# Autodesk Inventor assembly: CoreXY Motor Assembly Right for 4040 - V3
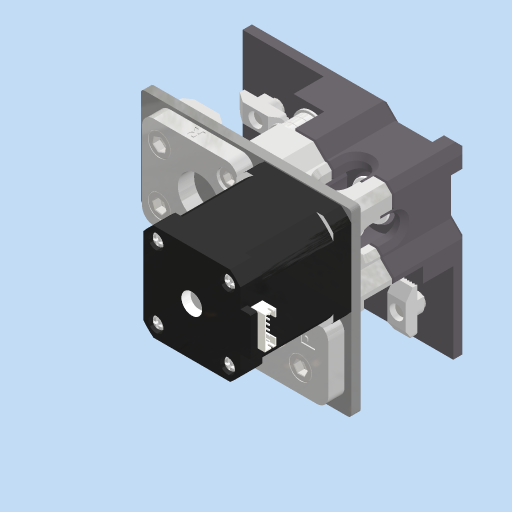
[picture p0: Inventor's stored thumbnail of the model, 512x512]
Saved by Autodesk Inventor 2023.2 (Build 272271000, 271)
## iProperties
Created: 2023-11-27
Part Number: CoreXY Motor Assembly Right for 4040 - V3
Document SubType Name: Assembly
Designer: Nils Bade
Author: Nils Bade
## Documents named in this file (17)
- C:\Users\nilsb\Documents\Inventor\Projektarbeit-Bade\RatRig_Bade\CoreXY Motor Assembly Right for 4040 - V3.iam
- C:\Users\nilsb\Documents\Inventor\Projektarbeit-Bade\RatRig_modified\Motor Plate Top for 4040.ipt
- C:\Users\nilsb\Documents\Inventor\Projektarbeit-Bade\RatRig_Standards\Nema 17 Stepper Motor - 48mm - 1.8degree_step, 76oz-in v1.ipt
- C:\Users\nilsb\Documents\Inventor\Projektarbeit-Bade\Schrauben\Cap Head Screw M3x35 v2.ipt
- C:\Users\nilsb\Documents\Inventor\Projektarbeit-Bade\RatRig_Standards\Timing Pulley - 2GT (2mm) - 20 Tooth - For 9mm Belt - 5mm Bo v1.ipt
- C:\Users\nilsb\Documents\Inventor\Projektarbeit-Bade\RatRig_modified\T-NUT - DropIn 4040 SERIES - M6.ipt
- C:\Users\nilsb\Documents\Inventor\Projektarbeit-Bade\Schrauben\Countersink Screw M6x14 v2.ipt
- C:\Users\nilsb\Documents\Inventor\Projektarbeit-Bade\Schrauben\Cap Head Screw M6x16.ipt
- C:\Users\nilsb\Documents\Inventor\Projektarbeit-Bade\RatRig_modified\xy Motor Support Left for 4040.ipt
- C:\Users\nilsb\Documents\Inventor\Projektarbeit-Bade\Schrauben\Cap Head Screw M5x40 v2.ipt
- C:\Users\nilsb\Documents\Inventor\Projektarbeit-Bade\RatRig_Standards\Hex Locking Nut - M5 v2.ipt
- C:\Users\nilsb\Documents\Inventor\Projektarbeit-Bade\RatRig_Standards\Mini Precision Shim - 8x5x1mm v2.ipt
- C:\Users\nilsb\Documents\Inventor\Projektarbeit-Bade\RatRig_Standards\Ball Bearing - F695ZZ v1.ipt
- C:\Users\nilsb\Documents\Inventor\Projektarbeit-Bade\RatRig_Standards\Ball Bearing - 695ZZ v1.ipt
- C:\Users\nilsb\Documents\Inventor\Projektarbeit-Bade\RatRig_modified\xy Motorcage Top Right for 4040 V2.ipt
- C:\Users\nilsb\Documents\Inventor\Projektarbeit-Bade\RatRig_modified\xy_motor_cage_bottom_right_v4.ipt
- C:\Users\nilsb\Documents\Inventor\Projektarbeit-Bade\RatRig_modified\xy Motor Support Right for 4040 extra.ipt
## Components (43 placed, 16 different names)
1. xy Motorcage Top Right for 4040 V2:2 — Passend:87
2. xy_motor_cage_bottom_right_v4:1 — Passend:87
3. Motor Plate Top for 4040:1 — Winkel:1, Passend:8, Passend:21, Passend:22, Passend:24, Passend:25, Winkel:5, Winkel:6, Winkel:7, Winkel:8, Passend:27, Passend:28, Passend:29, Passend:30, Passend:45, Passend:46, Passend:47, Passend:50, Passend:51, Passend:63, Passend:88, Passend:89, Passend:90, Passend:91, Passend:92, Passend:94
4. Nema 17 Stepper Motor - 48mm - 1.8degree_step, 76oz-in v1:1 — Winkel:1, Passend:8, Winkel:2, Passend:86
5. Cap Head Screw M3x35 v2:1
6. Cap Head Screw M3x35 v2:2
7. Cap Head Screw M3x35 v2:3
8. Cap Head Screw M3x35 v2:4
9. Timing Pulley - 2GT (2mm) - 20 Tooth - For 9mm Belt - 5mm Bo v1:1 — Winkel:2, Fluchtend:1, Passend:86
10. T-NUT - DROP IN TYPE FOR 40 SERIES - M6:1 — Passend:24, Winkel:7, Passend:28
11. T-NUT - DROP IN TYPE FOR 40 SERIES - M6:2 — Passend:25, Winkel:8, Passend:27
12. T-NUT - DROP IN TYPE FOR 40 SERIES - M6:3 — Passend:21, Winkel:5, Passend:30
13. T-NUT - DROP IN TYPE FOR 40 SERIES - M6:4 — Passend:22, Winkel:6, Passend:29, Passend:93
14. T-NUT - DROP IN TYPE FOR 40 SERIES - M6:5
15. T-NUT - DROP IN TYPE FOR 40 SERIES - M6:6
16. T-NUT - DROP IN TYPE FOR 40 SERIES - M6:7
17. Countersink Screw M6x14 v2:1
18. Countersink Screw M6x14 v2:2
19. Countersink Screw M6x14 v2:3
20. Cap Head Screw M6x16:1 — Passend:94, Passend:98
21. Cap Head Screw M6x16:2 — Passend:93, Passend:97
22. Cap Head Screw M6x16:3 — Passend:91, Passend:95
23. Cap Head Screw M6x16:4 — Passend:92, Passend:96
24. xy Motor Support Right for 4040 V2:1 — Passend:45, Passend:46, Passend:47, Passend:52, Passend:53, Passend:95, Passend:96
25. Cap Head Screw M5x40 v2:1 — Passend:50, Passend:53, Passend:54, Passend:58, Passend:59, Passend:67, Passend:69, Passend:71
26. Cap Head Screw M5x40 v2:2 — Passend:51, Passend:52, Passend:55, Passend:62, Passend:64, Passend:65, Passend:73, Passend:75, Passend:77, Passend:80, Passend:82, Passend:84
27. Hex Locking Nut - M5 v2:1 — Passend:55
28. Hex Locking Nut - M5 v2:2 — Passend:54
29. Mini Precision Shim - 8x5x1mm v2:1 — Passend:65, Passend:85
30. Mini Precision Shim - 8x5x1mm v2:2 — Passend:64, Passend:79, Passend:81
31. Mini Precision Shim - 8x5x1mm v2:3 — Passend:62, Passend:63, Passend:74
32. Mini Precision Shim - 8x5x1mm v2:4 — Passend:59, Passend:72
33. Mini Precision Shim - 8x5x1mm v2:5 — Passend:58, Passend:68
34. Ball Bearing - F695ZZ v1:1 — Passend:84, Passend:85, Fluchtend:1
35. Ball Bearing - F695ZZ v1:2 — Passend:77, Passend:78, Passend:79
36. Ball Bearing - F695ZZ v1:3 — Passend:71, Passend:72
37. Ball Bearing - F695ZZ v1:4 — Passend:80, Passend:81, Passend:83
38. Ball Bearing - F695ZZ v1:5 — Passend:73, Passend:74, Passend:76
39. Ball Bearing - F695ZZ v1:6 — Passend:67, Passend:68, Passend:70
40. Ball Bearing - 695ZZ v1:1 — Passend:82, Passend:83
41. Ball Bearing - 695ZZ v1:2 — Passend:75, Passend:76, Passend:78
42. Ball Bearing - 695ZZ v1:3 — Passend:69, Passend:70
43. xy Motor Support Right extra:1 — Passend:88, Passend:89, Passend:90, Passend:97, Passend:98
## Relationships (99: Mate 87, Angle 11, Flush 1)
- [Mate]: xy Motorcage Top Right for 4040 V2:2 ↔ xy_motor_cage_bottom_right_v4:1
- [Mate]: xy Motorcage Top Right for 4040 V2:2 ↔ xy_motor_cage_bottom_right_v4:1
- [Mate]: xy_motor_cage_bottom_right_v4:1 ↔ Motor Plate Top for 4040:1
- [Mate]: xy_motor_cage_bottom_right_v4:1 ↔ Motor Plate Top for 4040:1
- [Mate]: xy_motor_cage_bottom_right_v4:1 ↔ Motor Plate Top for 4040:1
- [Mate]: xy Motorcage Top Right for 4040 V2:2 ↔ Nema 17 Stepper Motor - 48mm - 1.8degree_step, 76oz-in v1:1
- Winkel:1 [Angle] (0 deg): Motor Plate Top for 4040:1 ↔ Nema 17 Stepper Motor - 48mm - 1.8degree_step, 76oz-in v1:1
- Passend:8 [Mate]: Motor Plate Top for 4040:1 ↔ Nema 17 Stepper Motor - 48mm - 1.8degree_step, 76oz-in v1:1
- [Mate]: xy Motorcage Top Right for 4040 V2:2 ↔ Cap Head Screw M3x35 v2:1
- [Mate]: xy Motorcage Top Right for 4040 V2:2 ↔ Cap Head Screw M3x35 v2:2
- [Mate]: xy Motorcage Top Right for 4040 V2:2 ↔ Cap Head Screw M3x35 v2:4
- [Mate]: xy Motorcage Top Right for 4040 V2:2 ↔ Cap Head Screw M3x35 v2:3
- [Mate]: xy Motorcage Top Right for 4040 V2:2 ↔ Cap Head Screw M3x35 v2:3
- [Mate]: xy Motorcage Top Right for 4040 V2:2 ↔ Cap Head Screw M3x35 v2:2
- [Mate]: xy Motorcage Top Right for 4040 V2:2 ↔ Cap Head Screw M3x35 v2:1
- [Mate]: xy Motorcage Top Right for 4040 V2:2 ↔ Cap Head Screw M3x35 v2:4
- Winkel:2 [Angle] (0 deg): Nema 17 Stepper Motor - 48mm - 1.8degree_step, 76oz-in v1:1 ↔ Timing Pulley - 2GT (2mm) - 20 Tooth - For 9mm Belt - 5mm Bo v1:1
- [Mate]: xy Motorcage Top Right for 4040 V2:2 ↔ T-NUT - DROP IN TYPE FOR 40 SERIES - M6:5
- [Mate]: xy Motorcage Top Right for 4040 V2:2 ↔ T-NUT - DROP IN TYPE FOR 40 SERIES - M6:6
- Passend:21 [Mate]: Motor Plate Top for 4040:1 ↔ T-NUT - DROP IN TYPE FOR 40 SERIES - M6:3
- Passend:22 [Mate]: Motor Plate Top for 4040:1 ↔ T-NUT - DROP IN TYPE FOR 40 SERIES - M6:4
- [Mate]: xy Motorcage Top Right for 4040 V2:2 ↔ T-NUT - DROP IN TYPE FOR 40 SERIES - M6:7
- Passend:24 [Mate]: Motor Plate Top for 4040:1 ↔ T-NUT - DROP IN TYPE FOR 40 SERIES - M6:1
- Passend:25 [Mate]: Motor Plate Top for 4040:1 ↔ T-NUT - DROP IN TYPE FOR 40 SERIES - M6:2
- [Angle] (0 deg): xy Motorcage Top Right for 4040 V2:2 ↔ T-NUT - DROP IN TYPE FOR 40 SERIES - M6:5
- [Angle] (0 deg): xy Motorcage Top Right for 4040 V2:2 ↔ T-NUT - DROP IN TYPE FOR 40 SERIES - M6:6
- Winkel:5 [Angle] (0 deg): Motor Plate Top for 4040:1 ↔ T-NUT - DROP IN TYPE FOR 40 SERIES - M6:3
- Winkel:6 [Angle] (0 deg): Motor Plate Top for 4040:1 ↔ T-NUT - DROP IN TYPE FOR 40 SERIES - M6:4
- Winkel:7 [Angle] (0 deg): Motor Plate Top for 4040:1 ↔ T-NUT - DROP IN TYPE FOR 40 SERIES - M6:1
- Winkel:8 [Angle] (0 deg): Motor Plate Top for 4040:1 ↔ T-NUT - DROP IN TYPE FOR 40 SERIES - M6:2
- [Angle] (0 deg): xy Motorcage Top Right for 4040 V2:2 ↔ T-NUT - DROP IN TYPE FOR 40 SERIES - M6:7
- [Mate] (4.5 mm): xy Motorcage Top Right for 4040 V2:2 ↔ T-NUT - DROP IN TYPE FOR 40 SERIES - M6:7
- Passend:27 [Mate] (4.5 mm): Motor Plate Top for 4040:1 ↔ T-NUT - DROP IN TYPE FOR 40 SERIES - M6:2
- Passend:28 [Mate] (4.5 mm): Motor Plate Top for 4040:1 ↔ T-NUT - DROP IN TYPE FOR 40 SERIES - M6:1
- Passend:29 [Mate] (4.5 mm): Motor Plate Top for 4040:1 ↔ T-NUT - DROP IN TYPE FOR 40 SERIES - M6:4
- Passend:30 [Mate] (4.5 mm): Motor Plate Top for 4040:1 ↔ T-NUT - DROP IN TYPE FOR 40 SERIES - M6:3
- [Mate] (4.5 mm): xy Motorcage Top Right for 4040 V2:2 ↔ T-NUT - DROP IN TYPE FOR 40 SERIES - M6:5
- [Mate] (4.5 mm): xy Motorcage Top Right for 4040 V2:2 ↔ T-NUT - DROP IN TYPE FOR 40 SERIES - M6:6
- [Mate]: xy Motorcage Top Right for 4040 V2:2 ↔ Countersink Screw M6x14 v2:3
- [Mate]: xy Motorcage Top Right for 4040 V2:2 ↔ Countersink Screw M6x14 v2:2
- [Mate]: xy Motorcage Top Right for 4040 V2:2 ↔ Countersink Screw M6x14 v2:1
- [Mate]: xy Motorcage Top Right for 4040 V2:2 ↔ Countersink Screw M6x14 v2:2
- [Mate]: xy Motorcage Top Right for 4040 V2:2 ↔ Countersink Screw M6x14 v2:1
- [Mate]: xy Motorcage Top Right for 4040 V2:2 ↔ Countersink Screw M6x14 v2:3
- Passend:45 [Mate]: Motor Plate Top for 4040:1 ↔ xy Motor Support Right for 4040 V2:1
- Passend:46 [Mate]: Motor Plate Top for 4040:1 ↔ xy Motor Support Right for 4040 V2:1
- Passend:47 [Mate]: Motor Plate Top for 4040:1 ↔ xy Motor Support Right for 4040 V2:1
- Passend:50 [Mate]: Motor Plate Top for 4040:1 ↔ Cap Head Screw M5x40 v2:1
- Passend:51 [Mate]: Motor Plate Top for 4040:1 ↔ Cap Head Screw M5x40 v2:2
- Passend:52 [Mate]: xy Motor Support Right for 4040 V2:1 ↔ Cap Head Screw M5x40 v2:2
- Passend:53 [Mate]: xy Motor Support Right for 4040 V2:1 ↔ Cap Head Screw M5x40 v2:1
- Passend:54 [Mate]: Cap Head Screw M5x40 v2:1 ↔ Hex Locking Nut - M5 v2:2
- Passend:55 [Mate]: Cap Head Screw M5x40 v2:2 ↔ Hex Locking Nut - M5 v2:1
- [Angle] (0 deg): xy Motorcage Top Right for 4040 V2:2 ↔ Hex Locking Nut - M5 v2:1
- [Angle] (0 deg): xy Motorcage Top Right for 4040 V2:2 ↔ Hex Locking Nut - M5 v2:2
- [Mate]: xy Motorcage Top Right for 4040 V2:2 ↔ Hex Locking Nut - M5 v2:1
- [Mate]: xy Motorcage Top Right for 4040 V2:2 ↔ Hex Locking Nut - M5 v2:2
- Passend:58 [Mate]: Cap Head Screw M5x40 v2:1 ↔ Mini Precision Shim - 8x5x1mm v2:5
- Passend:59 [Mate]: Cap Head Screw M5x40 v2:1 ↔ Mini Precision Shim - 8x5x1mm v2:4
- [Mate]: xy Motorcage Top Right for 4040 V2:2 ↔ Mini Precision Shim - 8x5x1mm v2:4
- [Mate]: xy_motor_cage_bottom_right_v4:1 ↔ Mini Precision Shim - 8x5x1mm v2:5
- Passend:62 [Mate]: Cap Head Screw M5x40 v2:2 ↔ Mini Precision Shim - 8x5x1mm v2:3
- Passend:63 [Mate]: Motor Plate Top for 4040:1 ↔ Mini Precision Shim - 8x5x1mm v2:3
- Passend:64 [Mate]: Cap Head Screw M5x40 v2:2 ↔ Mini Precision Shim - 8x5x1mm v2:2
- Passend:65 [Mate]: Cap Head Screw M5x40 v2:2 ↔ Mini Precision Shim - 8x5x1mm v2:1
- [Mate]: xy Motorcage Top Right for 4040 V2:2 ↔ Mini Precision Shim - 8x5x1mm v2:1
- Passend:67 [Mate]: Cap Head Screw M5x40 v2:1 ↔ Ball Bearing - F695ZZ v1:6
- Passend:68 [Mate]: Mini Precision Shim - 8x5x1mm v2:5 ↔ Ball Bearing - F695ZZ v1:6
- Passend:69 [Mate]: Cap Head Screw M5x40 v2:1 ↔ Ball Bearing - 695ZZ v1:3
- Passend:70 [Mate]: Ball Bearing - F695ZZ v1:6 ↔ Ball Bearing - 695ZZ v1:3
- Passend:71 [Mate]: Cap Head Screw M5x40 v2:1 ↔ Ball Bearing - F695ZZ v1:3
- Passend:72 [Mate]: Mini Precision Shim - 8x5x1mm v2:4 ↔ Ball Bearing - F695ZZ v1:3
- Passend:73 [Mate]: Cap Head Screw M5x40 v2:2 ↔ Ball Bearing - F695ZZ v1:5
- Passend:74 [Mate]: Mini Precision Shim - 8x5x1mm v2:3 ↔ Ball Bearing - F695ZZ v1:5
- Passend:75 [Mate]: Cap Head Screw M5x40 v2:2 ↔ Ball Bearing - 695ZZ v1:2
- Passend:76 [Mate]: Ball Bearing - F695ZZ v1:5 ↔ Ball Bearing - 695ZZ v1:2
- Passend:77 [Mate]: Cap Head Screw M5x40 v2:2 ↔ Ball Bearing - F695ZZ v1:2
- Passend:78 [Mate]: Ball Bearing - F695ZZ v1:2 ↔ Ball Bearing - 695ZZ v1:2
- Passend:79 [Mate]: Mini Precision Shim - 8x5x1mm v2:2 ↔ Ball Bearing - F695ZZ v1:2
- Passend:80 [Mate]: Cap Head Screw M5x40 v2:2 ↔ Ball Bearing - F695ZZ v1:4
- Passend:81 [Mate]: Mini Precision Shim - 8x5x1mm v2:2 ↔ Ball Bearing - F695ZZ v1:4
- Passend:82 [Mate]: Cap Head Screw M5x40 v2:2 ↔ Ball Bearing - 695ZZ v1:1
- Passend:83 [Mate]: Ball Bearing - F695ZZ v1:4 ↔ Ball Bearing - 695ZZ v1:1
- Passend:84 [Mate]: Cap Head Screw M5x40 v2:2 ↔ Ball Bearing - F695ZZ v1:1
- Passend:85 [Mate]: Mini Precision Shim - 8x5x1mm v2:1 ↔ Ball Bearing - F695ZZ v1:1
- Fluchtend:1 [Flush]: Timing Pulley - 2GT (2mm) - 20 Tooth - For 9mm Belt - 5mm Bo v1:1 ↔ Ball Bearing - F695ZZ v1:1
- Passend:86 [Mate]: Nema 17 Stepper Motor - 48mm - 1.8degree_step, 76oz-in v1:1 ↔ Timing Pulley - 2GT (2mm) - 20 Tooth - For 9mm Belt - 5mm Bo v1:1
- Passend:87 [Mate]: xy Motorcage Top Right for 4040 V2:2 ↔ xy_motor_cage_bottom_right_v4:1
- Passend:88 [Mate]: Motor Plate Top for 4040:1 ↔ xy Motor Support Right extra:1
- Passend:89 [Mate]: Motor Plate Top for 4040:1 ↔ xy Motor Support Right extra:1
- Passend:90 [Mate]: Motor Plate Top for 4040:1 ↔ xy Motor Support Right extra:1
- Passend:91 [Mate]: Motor Plate Top for 4040:1 ↔ Cap Head Screw M6x16:3
- Passend:92 [Mate]: Motor Plate Top for 4040:1 ↔ Cap Head Screw M6x16:4
- Passend:93 [Mate]: T-NUT - DROP IN TYPE FOR 40 SERIES - M6:4 ↔ Cap Head Screw M6x16:2
- Passend:94 [Mate]: Motor Plate Top for 4040:1 ↔ Cap Head Screw M6x16:1
- Passend:95 [Mate]: Cap Head Screw M6x16:3 ↔ xy Motor Support Right for 4040 V2:1
- Passend:96 [Mate]: Cap Head Screw M6x16:4 ↔ xy Motor Support Right for 4040 V2:1
- Passend:97 [Mate]: Cap Head Screw M6x16:2 ↔ xy Motor Support Right extra:1
- Passend:98 [Mate]: Cap Head Screw M6x16:1 ↔ xy Motor Support Right extra:1
